# Autodesk Inventor assembly: Lifter Super Structure
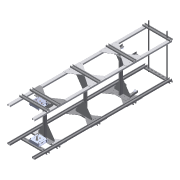
[picture p0: Inventor's stored thumbnail of the model, 180x180]
Saved by Autodesk Inventor 2015 (Build 190159000, 159)
## iProperties
Created: 2015-01-24
Part Number: Lifter Super Structure
Document SubType Name: Assembly
Designer: Peter
Author: Peter
## Documents named in this file (3)
- C:\Users\Noah\Desktop\FIRST-Team-1719-CAD-Team\2015 Robot CAD\Lifter Super Structure\Lifter Super Structure.iam
- C:\Users\Noah\Desktop\FIRST-Team-1719-CAD-Team\2015 Robot CAD\Lifter Super Structure\Tower\Tower Assembly.iam
- C:\Users\Noah\Desktop\FIRST-Team-1719-CAD-Team\2015 Robot CAD\Lifter Super Structure\Tower\Brackets\super3.ipt
## Components (9 placed, 2 different names)
1. Tower Assembly:1 [sub-assembly] — Mate:1, Angle:1, Mate:2, Flush:1, Flush:2, Mate:3, Mate:4, Mate:5, Flush:3, Mate:6, Mate:7, Flush:4, Mate:8, Mate:9, Mate:10, Flush:5, Flush:6, Mate:11, Mate:12, Mate:13, Mate:14, Flush:7, Flush:8, Mate:15, Mate:16
2. super3:1 — Mate:1, Angle:1, Mate:2, Flush:1
3. super3:2 — Flush:2, Mate:3, Mate:4
4. super3:3 — Mate:7, Flush:4, Mate:8
5. super3:4 — Mate:5, Flush:3, Mate:6
6. super3:5 — Mate:10, Flush:5, Mate:12
7. super3:6 — Mate:14, Flush:8, Mate:15
8. super3:7 — Mate:13, Flush:7, Mate:16
9. super3:8 — Mate:9, Flush:6, Mate:11
## Relationships (25: Mate 16, Flush 8, Angle 1)
- Mate:1: Tower Assembly:1 ↔ super3:1
- Angle:1 (0 deg): Tower Assembly:1 ↔ super3:1
- Mate:2 (2.0955 mm): Tower Assembly:1 ↔ super3:1
- Flush:1: Tower Assembly:1 ↔ super3:1
- Flush:2: Tower Assembly:1 ↔ super3:2
- Mate:3: Tower Assembly:1 ↔ super3:2
- Mate:4 (2.0955 mm): Tower Assembly:1 ↔ super3:2
- Mate:5: Tower Assembly:1 ↔ super3:4
- Flush:3: Tower Assembly:1 ↔ super3:4
- Mate:6 (2.0955 mm): Tower Assembly:1 ↔ super3:4
- Mate:7: Tower Assembly:1 ↔ super3:3
- Flush:4: Tower Assembly:1 ↔ super3:3
- Mate:8 (2.0955 mm): Tower Assembly:1 ↔ super3:3
- Mate:9: Tower Assembly:1 ↔ super3:8
- Mate:10: Tower Assembly:1 ↔ super3:5
- Flush:5: Tower Assembly:1 ↔ super3:5
- Flush:6: Tower Assembly:1 ↔ super3:8
- Mate:11 (2.0955 mm): Tower Assembly:1 ↔ super3:8
- Mate:12 (2.0955 mm): Tower Assembly:1 ↔ super3:5
- Mate:13: Tower Assembly:1 ↔ super3:7
- Mate:14: Tower Assembly:1 ↔ super3:6
- Flush:7: Tower Assembly:1 ↔ super3:7
- Flush:8: Tower Assembly:1 ↔ super3:6
- Mate:15 (2.0955 mm): Tower Assembly:1 ↔ super3:6
- Mate:16 (2.0955 mm): Tower Assembly:1 ↔ super3:7
